# Autodesk Inventor assembly: Gobilda bevel gears + 8mm REX hyper hub
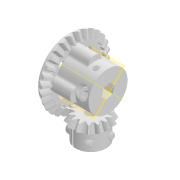
[picture p0: Inventor's stored thumbnail of the model, 180x180]
Saved by Autodesk Inventor 2020 (Build 240168000, 168)
## iProperties
Created: 2020-02-29
Part Number: Gobilda bevel gears + 8mm REX hyper hub
Document SubType Name: Assembly
Designer: ball
Author: ball
## Documents named in this file (4)
- C:\FTC\FTC8863CAD\2019 Robot\Generic Parts\Gobilda bevel gears + 8mm REX hyper hub.iam
- C:\FTC\FTC8863CAD\GoBilda\3204 Parts\3204-0002-0001 assembly.iam
- C:\FTC\FTC8863CAD\GoBilda\1310 Parts\1310-0016-4008 assembly.ipt
- C:\FTC\FTC8863CAD\StepLibraries\Screws\M4 x 12 SOCKET HEAD CAP SCREW.ipt
## Components (6 placed, 3 different names)
1. 3204-0002-0001 assembly:1 [sub-assembly] — Mate:1, Mate:2, Mate:3, Mate:4, Mate:5, Mate:6, Mate:7, Mate:8, Mate:9, Mate:10, Mate:11, Mate:12
2. 1310-0016-4008 assembly:1 — Mate:1, Mate:2, Mate:3, Mate:4
3. M4 x 12 SOCKET HEAD CAP SCREW:1 — Mate:5, Mate:11
4. M4 x 12 SOCKET HEAD CAP SCREW:2 — Mate:6, Mate:12
5. M4 x 12 SOCKET HEAD CAP SCREW:3 — Mate:7, Mate:10
6. M4 x 12 SOCKET HEAD CAP SCREW:4 — Mate:8, Mate:9
## Relationships (12: Mate 12)
- Mate:1: 3204-0002-0001 assembly:1 ↔ 1310-0016-4008 assembly:1
- Mate:2: 3204-0002-0001 assembly:1 ↔ 1310-0016-4008 assembly:1
- Mate:3: 3204-0002-0001 assembly:1 ↔ 1310-0016-4008 assembly:1
- Mate:4: 3204-0002-0001 assembly:1 ↔ 1310-0016-4008 assembly:1
- Mate:5: 3204-0002-0001 assembly:1 ↔ M4 x 12 SOCKET HEAD CAP SCREW:1
- Mate:6: 3204-0002-0001 assembly:1 ↔ M4 x 12 SOCKET HEAD CAP SCREW:2
- Mate:7: 3204-0002-0001 assembly:1 ↔ M4 x 12 SOCKET HEAD CAP SCREW:3
- Mate:8: 3204-0002-0001 assembly:1 ↔ M4 x 12 SOCKET HEAD CAP SCREW:4
- Mate:9: 3204-0002-0001 assembly:1 ↔ M4 x 12 SOCKET HEAD CAP SCREW:4
- Mate:10: 3204-0002-0001 assembly:1 ↔ M4 x 12 SOCKET HEAD CAP SCREW:3
- Mate:11: 3204-0002-0001 assembly:1 ↔ M4 x 12 SOCKET HEAD CAP SCREW:1
- Mate:12: 3204-0002-0001 assembly:1 ↔ M4 x 12 SOCKET HEAD CAP SCREW:2
